# Autodesk Inventor assembly: Motor_64_no_idle_ver
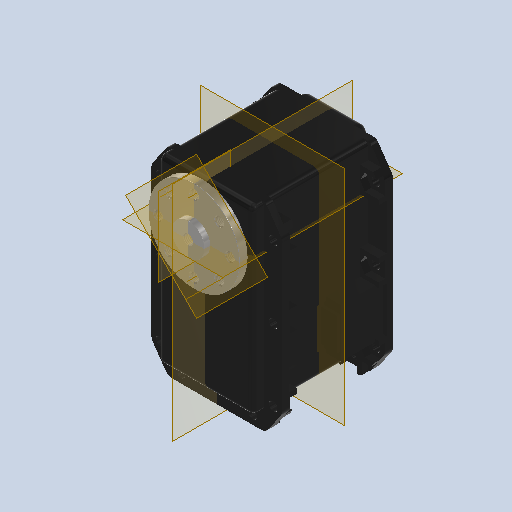
[picture p0: Inventor's stored thumbnail of the model, 512x512]
Saved by Autodesk Inventor 2024.3 (Build 283343000, 343)
## iProperties
Created: 2024-09-06
Part Number: Motor_64_no_idle_ver
Document SubType Name: Assembly
Designer: gretc
Author: gretc
## Documents named in this file (3)
- C:\Users\USER\Desktop\로빛 예비인턴\(git)19기 이원준 격투로봇 설계파일\motor\Motor_64_no_idle_ver.iam
- C:\Users\USER\Desktop\로빛 예비인턴\예비인턴 격투로봇 설계 프로젝트\격투로봇 백업 2\다이나믹셀\MX-64T.ipt
- C:\Users\USER\Desktop\로빛 예비인턴\예비인턴 격투로봇 설계 프로젝트\혼\64-106Horn.ipt
## Components (2 placed, 2 different names)
1. MX-64T:1 — 삽입:1, 각도:1
2. 64-106Horn:1 — 삽입:1, 메이트:1, 메이트:2
## Relationships (6: Mate 4, Insert 1, Angle 1)
- 삽입:1 [Insert] (0.5 mm): MX-64T:1 ↔ 64-106Horn:1
- 메이트:1 [Mate]: 64-106Horn:1
- 메이트:2 [Mate]: 64-106Horn:1
- 메이트:3 [Mate]
- 메이트:4 [Mate]
- 각도:1 [Angle] (90 deg): MX-64T:1
